# Autodesk Inventor assembly: tank tread
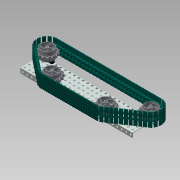
[picture p0: Inventor's stored thumbnail of the model, 180x180]
Saved by Autodesk Inventor 2013 (Build 170138000, 138)
## iProperties
Created: 2013-02-04
Part Number: tank tread
Document SubType Name: Assembly
Designer: NNolte
Author: NNolte
## Documents named in this file (6)
- F:\POE\VEX 2013\Chain Example\tank tread.iam
- F:\POE\VEX 2013\C-Channel 1x5x1x25 Hole.ipt
- F:\POE\VEX 2013\Bearing Flat.ipt
- F:\POE\VEX 2013\Tank Tread Drive Wheel.ipt
- F:\POE\VEX 2013\Chain Example\tank tread path.ipt
- F:\POE\VEX 2013\Link - Tank Tread.ipt
## Components (88 placed, 5 different names)
1. C-Channel 1x5x1x25 Hole:1 — Insert:1, Insert:2, Insert:3, Insert:4, Insert:5, Insert:6, Insert:7, Insert:8
2. Bearing Flat:1 — Insert:1, Insert:2, Insert:12
3. Bearing Flat:2 — Insert:7, Insert:8, Insert:15
4. Bearing Flat:3 — Insert:5, Insert:6, Insert:14
5. Bearing Flat:4 — Insert:3, Insert:4, Insert:13
6. Tank Tread Drive Wheel:1 — Flush:1, Flush:2, Insert:12
7. Tank Tread Drive Wheel:2 — Insert:13
8. Tank Tread Drive Wheel:3 — Insert:14
9. Tank Tread Drive Wheel:4 — Insert:15
10. tank tread path:1 — Flush:1, Flush:2, Mate:1, Angle:2, Mate:2
11. Link - Tank Tread:1 — Mate:1, Angle:2, Mate:2
12. Link - Tank Tread:2
13. Link - Tank Tread:3
14. Link - Tank Tread:4
15. Link - Tank Tread:5
16. Link - Tank Tread:6
17. Link - Tank Tread:7
18. Link - Tank Tread:8
19. Link - Tank Tread:9
20. Link - Tank Tread:10
21. Link - Tank Tread:11
22. Link - Tank Tread:12
23. Link - Tank Tread:13
24. Link - Tank Tread:14
25. Link - Tank Tread:15
26. Link - Tank Tread:16
27. Link - Tank Tread:17
28. Link - Tank Tread:18
29. Link - Tank Tread:19
30. Link - Tank Tread:20
31. Link - Tank Tread:21
32. Link - Tank Tread:22
33. Link - Tank Tread:23
34. Link - Tank Tread:24
35. Link - Tank Tread:25
36. Link - Tank Tread:26
37. Link - Tank Tread:27
38. Link - Tank Tread:28
39. Link - Tank Tread:29
40. Link - Tank Tread:30
41. Link - Tank Tread:31
42. Link - Tank Tread:32
43. Link - Tank Tread:33
44. Link - Tank Tread:34
45. Link - Tank Tread:35
46. Link - Tank Tread:36
47. Link - Tank Tread:37
48. Link - Tank Tread:38
49. Link - Tank Tread:39
50. Link - Tank Tread:40
51. Link - Tank Tread:41
52. Link - Tank Tread:42
53. Link - Tank Tread:43
54. Link - Tank Tread:44
55. Link - Tank Tread:45
56. Link - Tank Tread:46
57. Link - Tank Tread:47
58. Link - Tank Tread:48
59. Link - Tank Tread:49
60. Link - Tank Tread:50
61. Link - Tank Tread:51
62. Link - Tank Tread:52
63. Link - Tank Tread:53
64. Link - Tank Tread:54
65. Link - Tank Tread:55
66. Link - Tank Tread:56
67. Link - Tank Tread:57
68. Link - Tank Tread:58
69. Link - Tank Tread:59
70. Link - Tank Tread:60
71. Link - Tank Tread:61
72. Link - Tank Tread:62
73. Link - Tank Tread:63
74. Link - Tank Tread:64
75. Link - Tank Tread:65
76. Link - Tank Tread:66
77. Link - Tank Tread:67
78. Link - Tank Tread:68
79. Link - Tank Tread:69
80. Link - Tank Tread:70
81. Link - Tank Tread:71
82. Link - Tank Tread:72
83. Link - Tank Tread:73
84. Link - Tank Tread:74
85. Link - Tank Tread:75
86. Link - Tank Tread:76
87. Link - Tank Tread:77
88. Link - Tank Tread:78
## Component patterns: (78 elements, first: Link - Tank Tread:1)
## Relationships (17: Insert 12, Flush 2, Mate 2, Angle 1)
- Flush:1: Tank Tread Drive Wheel:1 ↔ tank tread path:1
- Flush:2: Tank Tread Drive Wheel:1 ↔ tank tread path:1
- Mate:1: tank tread path:1 ↔ Link - Tank Tread:1
- Angle:2 (270 deg): tank tread path:1 ↔ Link - Tank Tread:1
- Mate:2: tank tread path:1 ↔ Link - Tank Tread:1
- Insert:1: C-Channel 1x5x1x25 Hole:1 ↔ Bearing Flat:1
- Insert:2: C-Channel 1x5x1x25 Hole:1 ↔ Bearing Flat:1
- Insert:3: C-Channel 1x5x1x25 Hole:1 ↔ Bearing Flat:4
- Insert:4: C-Channel 1x5x1x25 Hole:1 ↔ Bearing Flat:4
- Insert:5: C-Channel 1x5x1x25 Hole:1 ↔ Bearing Flat:3
- Insert:6: C-Channel 1x5x1x25 Hole:1 ↔ Bearing Flat:3
- Insert:7: C-Channel 1x5x1x25 Hole:1 ↔ Bearing Flat:2
- Insert:8: C-Channel 1x5x1x25 Hole:1 ↔ Bearing Flat:2
- Insert:12: Bearing Flat:1 ↔ Tank Tread Drive Wheel:1
- Insert:13: Bearing Flat:4 ↔ Tank Tread Drive Wheel:2
- Insert:14: Bearing Flat:3 ↔ Tank Tread Drive Wheel:3
- Insert:15: Bearing Flat:2 ↔ Tank Tread Drive Wheel:4
